# Autodesk Inventor assembly: Bản vẽ mô tả 3D - Giá đỡ động cơ
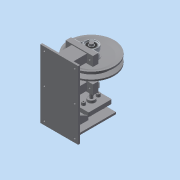
[picture p0: Inventor's stored thumbnail of the model, 180x180]
Saved by Autodesk Inventor 2018 (Build 220112000, 112)
## iProperties
Created: 2020-10-11
Part Number: Bản vẽ mô tả 3D - Giá đỡ động cơ
Document SubType Name: Assembly
Designer: ASUS
Author: ASUS
## Documents named in this file (7)
- E:\CTU\Skylight\Bản vẽ\Bản vẽ Giếng Trời Tự Động\Bản vẽ 3D\Bản vẽ mô tả 3D - Giá đỡ động cơ.iam
- E:\CTU\Skylight\Bản vẽ\Bản vẽ Giếng Trời Tự Động\Bản vẽ 3D\Giá đỡ động cơ + trục\Giá đỡ động cơ.ipt
- E:\CTU\Skylight\Bản vẽ\Bản vẽ Giếng Trời Tự Động\Bản vẽ 3D\Linh kiện khác\Gối đỡ\Gối đỡ KP000 - d10mm.ipt
- E:\CTU\Skylight\Bản vẽ\Bản vẽ Giếng Trời Tự Động\Bản vẽ 3D\Linh kiện khác\Động cơ 775 + Giảm tốc\Động cơ 775 + Giảm tốc.iam
- E:\CTU\Skylight\Bản vẽ\Bản vẽ Giếng Trời Tự Động\Bản vẽ 3D\Giá đỡ động cơ + trục\Trục 10.ipt
- E:\CTU\Skylight\Bản vẽ\Bản vẽ Giếng Trời Tự Động\Bản vẽ 3D\Linh kiện khác\Bánh đà\bánh đà.ipt
- E:\CTU\Skylight\Bản vẽ\Bản vẽ Giếng Trời Tự Động\Bản vẽ 3D\Linh kiện khác\Khớp nối\Khớp nối cứng.ipt
## Components (7 placed, 6 different names)
1. Giá đỡ động cơ:1 — Mate:1, Mate:2, Mate:3, Mate:4, Mate:5, Mate:6, Mate:7, Mate:8, Mate:9
2. Động cơ 775 + Giảm tốc:1 [sub-assembly] — Mate:7, Mate:8, Mate:9, Mate:13
3. Gối đỡ KP000 - d10mm:1 — Mate:1, Mate:2, Mate:3
4. Gối đỡ KP000 - d10mm:2 — Mate:4, Mate:5, Mate:6, Mate:10, Flush:1
5. Trục 10:1 — Mate:10, Flush:1, Mate:11, Flush:2, Mate:12
6. bánh đà:1 — Mate:11, Flush:2
7. Khớp nối cứng:1 — Mate:12, Mate:13
## Relationships (15: Mate 13, Flush 2)
- Mate:1: Giá đỡ động cơ:1 ↔ Gối đỡ KP000 - d10mm:1
- Mate:2: Giá đỡ động cơ:1 ↔ Gối đỡ KP000 - d10mm:1
- Mate:3: Giá đỡ động cơ:1 ↔ Gối đỡ KP000 - d10mm:1
- Mate:4: Giá đỡ động cơ:1 ↔ Gối đỡ KP000 - d10mm:2
- Mate:5: Giá đỡ động cơ:1 ↔ Gối đỡ KP000 - d10mm:2
- Mate:6: Giá đỡ động cơ:1 ↔ Gối đỡ KP000 - d10mm:2
- Mate:7: Giá đỡ động cơ:1 ↔ Động cơ 775 + Giảm tốc:1
- Mate:8: Giá đỡ động cơ:1 ↔ Động cơ 775 + Giảm tốc:1
- Mate:9: Giá đỡ động cơ:1 ↔ Động cơ 775 + Giảm tốc:1
- Mate:10: Gối đỡ KP000 - d10mm:2 ↔ Trục 10:1
- Flush:1 (-5 mm): Gối đỡ KP000 - d10mm:2 ↔ Trục 10:1
- Mate:11: Trục 10:1 ↔ bánh đà:1
- Flush:2: Trục 10:1 ↔ bánh đà:1
- Mate:12: Trục 10:1 ↔ Khớp nối cứng:1
- Mate:13 (-10 mm): Động cơ 775 + Giảm tốc:1 ↔ Khớp nối cứng:1
